# Autodesk Inventor assembly: Chassis
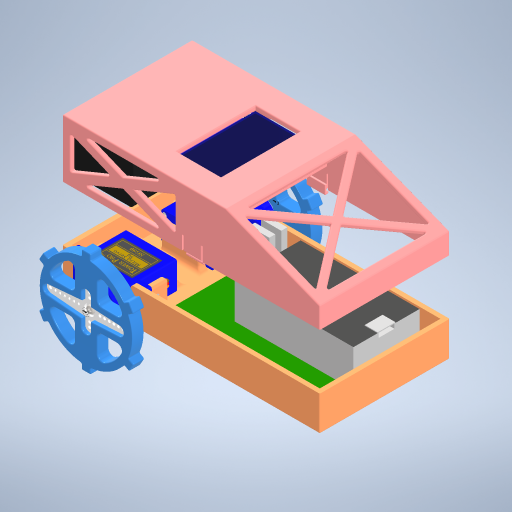
[picture p0: Inventor's stored thumbnail of the model, 512x512]
Saved by Autodesk Inventor 2024 (Build 280153000, 153)
## iProperties
Created: 2024-05-21
Part Number: Chassis
Document SubType Name: Assembly
Designer: andre
Author: andre
## Documents named in this file (8)
- C:\Users\andre\Documents\GitHub\Handshake\Hardware\Chassis.iam
- C:\Users\andre\Downloads\SG90 - Micro Servo 9g - Tower Pro\SG90 - Micro Servo 9g - Tower Pro.iam
- C:\Users\andre\Documents\GitHub\Handshake\Hardware\PCBModel.ipt
- C:\Users\andre\Documents\GitHub\Handshake\Hardware\case1btm.ipt
- C:\Users\andre\Documents\GitHub\Handshake\Hardware\battery.ipt
- C:\Users\andre\Documents\GitHub\Handshake\Hardware\case1top.ipt
- C:\Users\andre\Downloads\sh1106-1-3-1.snapshot.2\Oled SH1106\Oled SH1106.ipt
- C:\Users\andre\Documents\GitHub\Handshake\Hardware\wheel1.ipt
## Components (9 placed, 7 different names)
1. SG90 - Micro Servo 9g - Tower Pro:1 [sub-assembly] — Flush:1, Flush:2, Mate:5, Mate:6, Mate:15, Mate:16
2. SG90 - Micro Servo 9g - Tower Pro:2 [sub-assembly] — Flush:1, Flush:2, Mate:3, Mate:4, Mate:13, Mate:14
3. PCBModel:1 — Mate:1, Mate:2
4. case1btm:1 — Mate:1, Mate:2, Mate:3, Mate:4, Mate:5, Mate:6, Mate:12
5. battery:1 — Mate:7, Mate:8
6. case1top:1 — Mate:7, Mate:8, Mate:9, Mate:10, Mate:11, Mate:12
7. Oled SH1106:1 — Mate:9, Mate:10, Mate:11
8. wheel1:1 — Mate:13, Mate:14
9. wheel1:2 — Mate:15, Mate:16
## Relationships (18: Mate 16, Flush 2)
- Mate:1: PCBModel:1 ↔ case1btm:1
- Mate:2: PCBModel:1 ↔ case1btm:1
- Flush:1: SG90 - Micro Servo 9g - Tower Pro:1 ↔ SG90 - Micro Servo 9g - Tower Pro:2
- Flush:2: SG90 - Micro Servo 9g - Tower Pro:1 ↔ SG90 - Micro Servo 9g - Tower Pro:2
- Mate:3: SG90 - Micro Servo 9g - Tower Pro:2 ↔ case1btm:1
- Mate:4: SG90 - Micro Servo 9g - Tower Pro:2 ↔ case1btm:1
- Mate:5: SG90 - Micro Servo 9g - Tower Pro:1 ↔ case1btm:1
- Mate:6: SG90 - Micro Servo 9g - Tower Pro:1 ↔ case1btm:1
- Mate:7 (0.5 mm): battery:1 ↔ case1top:1
- Mate:8 (0.5 mm): battery:1 ↔ case1top:1
- Mate:9: case1top:1 ↔ Oled SH1106:1
- Mate:10 (-0.2 mm): case1top:1 ↔ Oled SH1106:1
- Mate:11: case1top:1 ↔ Oled SH1106:1
- Mate:12 (2 mm): case1btm:1 ↔ case1top:1
- Mate:13: SG90 - Micro Servo 9g - Tower Pro:2 ↔ wheel1:1
- Mate:14: SG90 - Micro Servo 9g - Tower Pro:2 ↔ wheel1:1
- Mate:15: SG90 - Micro Servo 9g - Tower Pro:1 ↔ wheel1:2
- Mate:16: SG90 - Micro Servo 9g - Tower Pro:1 ↔ wheel1:2
